# Autodesk Inventor assembly: FrontOdomPod
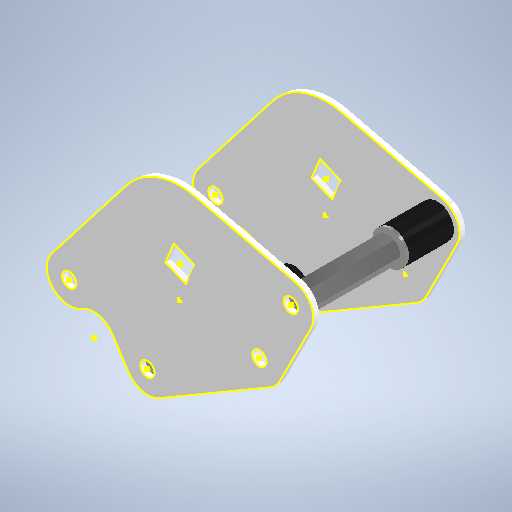
[picture p0: Inventor's stored thumbnail of the model, 512x512]
Saved by Autodesk Inventor 2025.2 (Build 292293000, 293)
## iProperties
Created: 2025-03-23
Part Number: FrontOdomPod
Document SubType Name: Assembly
Designer: roejo
Author: roejo
## Documents named in this file (9)
- C:\1629X-7700R-Worlds-Bot\Bot 1\FrontOdomPod.iam
- C:\1629X-7700R-Worlds-Bot\Bot 1\Plastic\Odom\Front Horizontal Odom Pod nonRot Side.ipt
- C:\1629X-7700R-Worlds-Bot\Bot 1\Plastic\Odom\Front Horizontal Odom Pod Rot Side.ipt
- C:\1629X-7700R-Worlds-Bot\VEX-CAD-Inventor-1.4.2\Motion\Spacers\Washer Steel\SWasher .375 OD x .031250.ipt
- C:\1629X-7700R-Worlds-Bot\VEX-CAD-Inventor-1.4.2\Motion\Spacers\Washer Steel.ipt
- C:\1629X-7700R-Worlds-Bot\VEX-CAD-Inventor-1.4.2\Structure\Standoff\Standoff 1.00.ipt
- C:\1629X-7700R-Worlds-Bot\VEX-CAD-Inventor-1.4.2\Structure\Standoff.ipt
- C:\1629X-7700R-Worlds-Bot\VEX-CAD-Inventor-1.4.2\Motion\Spacers\Spacer Nylon .375 OD\NSpacer .375 OD x .500.ipt
- C:\1629X-7700R-Worlds-Bot\VEX-CAD-Inventor-1.4.2\Motion\Spacers\Spacer Nylon .375 OD.ipt
## Components (10 placed, 5 different names)
1. Front Horizontal Odom Pod nonRot Side:1 — Insert:5
2. Front Horizontal Odom Pod Rot Side:1 — Insert:1, Insert:9
3. SWasher .375 OD x .031250:1 — Insert:3, Insert:4
4. SWasher .375 OD x .031250:2 — Insert:1, Insert:2
5. Standoff 1.00:1 — Insert:2, Insert:3
6. NSpacer .375 OD x .500:1 — Insert:4, Insert:5
7. SWasher .375 OD x .031250:3
8. SWasher .375 OD x .031250:4 — Insert:9
9. Standoff 1.00:2
10. NSpacer .375 OD x .500:2
## Relationships (9: Insert 9)
- Insert:1: Front Horizontal Odom Pod Rot Side:1 ↔ SWasher .375 OD x .031250:2
- Insert:2: SWasher .375 OD x .031250:2 ↔ Standoff 1.00:1
- Insert:3: SWasher .375 OD x .031250:1 ↔ Standoff 1.00:1
- Insert:4: SWasher .375 OD x .031250:1 ↔ NSpacer .375 OD x .500:1
- Insert:5: Front Horizontal Odom Pod nonRot Side:1 ↔ NSpacer .375 OD x .500:1
- [Insert]: SWasher .375 OD x .031250:4 ↔ Standoff 1.00:2
- [Insert]: SWasher .375 OD x .031250:3 ↔ Standoff 1.00:2
- [Insert]: SWasher .375 OD x .031250:3 ↔ NSpacer .375 OD x .500:2
- Insert:9: Front Horizontal Odom Pod Rot Side:1 ↔ SWasher .375 OD x .031250:4
## Named parameters: d5_d1 = 0 mm, d6_d2 = 0 mm, d7_d3 = 0 mm
